# Autodesk Inventor assembly: cube sat
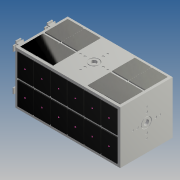
[picture p0: Inventor's stored thumbnail of the model, 180x180]
Saved by Autodesk Inventor 2017 SP1 (Build 210196100, 196)
## iProperties
Part Number: cube sat
Material: Generico
Document SubType Name: Assembly
Designer: De Grandis Leonardo
Author: De Grandis Leonardo
## Documents named in this file (8)
- E:\MATERIALE DA CARICARE\cube sat.iam
- C:\Users\Leonardo\3D Objects\struttura satellitino.ipt
- C:\Users\Leonardo\3D Objects\lente fotocamera.ipt
- C:\Users\Leonardo\3D Objects\laser 1.ipt
- C:\Users\Leonardo\3D Objects\laser 2.ipt
- C:\Users\Leonardo\3D Objects\pannello solare.ipt
- C:\Users\Leonardo\3D Objects\pannello solare_CPY.ipt
- C:\Users\Leonardo\3D Objects\pannello solare_CPY1.ipt
## Components (49 placed, 7 different names)
1. struttura satellitino:1 — Coincidente:1, Coincidente:2, Coincidente:3, Coincidente:4, Coincidente:5, Coincidente:6, Coincidente:7, Coincidente:8, Coincidente:9, Coincidente:10, Coincidente:11, Coincidente:12, Coincidente:13, Coincidente:17, Coincidente:18, Coincidente:19, Coincidente:20, Coincidente:21, Coincidente:22, Coincidente:23, Coincidente:24, Coincidente:25, Coincidente:26, Coincidente:27, Coincidente:28, Coincidente:29, Coincidente:30, Coincidente:31, Coincidente:32, Coincidente:33, Coincidente:34, Coincidente:35, Coincidente:36, Coincidente:37, Coincidente:38, Coincidente:39, Coincidente:40, Coincidente:41
2. lente fotocamera:1 — Coincidente:3
3. laser 1:1 — Coincidente:4, Coincidente:5
4. laser 1:2 — Coincidente:6, Coincidente:7
5. laser 2:1 — Coincidente:8, Coincidente:9
6. pannello solare:1 — Coincidente:10, Coincidente:11, Coincidente:12, Coincidente:13
7. pannello solare:2 — Coincidente:17, Coincidente:18, Coincidente:19
8. pannello solare:3
9. pannello solare:4
10. pannello solare:5
11. pannello solare:6
12. pannello solare:7
13. pannello solare:8
14. pannello solare:9
15. pannello solare:10
16. pannello solare:11
17. pannello solare:12
18. pannello solare_CPY:1 — Coincidente:20, Coincidente:22, Coincidente:23
19. pannello solare_CPY:2 — Coincidente:24, Coincidente:25
20. pannello solare_CPY:3
21. pannello solare_CPY:4 — Coincidente:21
22. pannello solare_CPY:5
23. pannello solare_CPY:6
24. pannello solare_CPY:7
25. pannello solare_CPY:8
26. pannello solare_CPY:9
27. pannello solare_CPY:10
28. pannello solare_CPY:11
29. pannello solare_CPY:12
30. pannello solare_CPY1:1
31. pannello solare_CPY1:2
32. pannello solare_CPY1:3
33. pannello solare_CPY1:4
34. pannello solare_CPY1:5
35. pannello solare_CPY1:6
36. pannello solare_CPY1:7
37. pannello solare_CPY1:8
38. pannello solare_CPY1:9
39. pannello solare_CPY1:10 — Coincidente:31
40. pannello solare_CPY1:11 — Coincidente:27, Coincidente:29, Coincidente:30
41. pannello solare_CPY1:12 — Coincidente:26, Coincidente:28
42. pannello solare:16 — Coincidente:32, Coincidente:33
43. pannello solare:15 — Coincidente:34, Coincidente:35
44. pannello solare:13 — Coincidente:36, Coincidente:37, Coincidente:38
45. pannello solare:17 — Coincidente:39, Coincidente:40, Coincidente:41
46. pannello solare:18
47. pannello solare:19
48. pannello solare:20
49. pannello solare:21
## Component patterns: (6 elements, first: pannello solare:1 + pannello solare:2), (6 elements, first: pannello solare_CPY:1 + pannello solare_CPY:2), (6 elements, first: pannello solare_CPY1:1 + pannello solare_CPY1:2), (2 elements, first: pannello solare:16 + pannello solare:15 + pannello solare:13 + pannello solare:17)
## Relationships (38: Mate 38)
- Coincidente:1 [Mate]: struttura satellitino:1
- Coincidente:2 [Mate]: struttura satellitino:1
- Coincidente:3 [Mate]: struttura satellitino:1 ↔ lente fotocamera:1
- Coincidente:4 [Mate]: struttura satellitino:1 ↔ laser 1:1
- Coincidente:5 [Mate]: struttura satellitino:1 ↔ laser 1:1
- Coincidente:6 [Mate]: struttura satellitino:1 ↔ laser 1:2
- Coincidente:7 [Mate]: struttura satellitino:1 ↔ laser 1:2
- Coincidente:8 [Mate]: struttura satellitino:1 ↔ laser 2:1
- Coincidente:9 [Mate]: struttura satellitino:1 ↔ laser 2:1
- Coincidente:10 [Mate]: struttura satellitino:1 ↔ pannello solare:1
- Coincidente:11 [Mate]: struttura satellitino:1 ↔ pannello solare:1
- Coincidente:12 [Mate]: struttura satellitino:1 ↔ pannello solare:1
- Coincidente:13 [Mate]: struttura satellitino:1 ↔ pannello solare:1
- Coincidente:17 [Mate]: struttura satellitino:1 ↔ pannello solare:2
- Coincidente:18 [Mate]: struttura satellitino:1 ↔ pannello solare:2
- Coincidente:19 [Mate]: struttura satellitino:1 ↔ pannello solare:2
- Coincidente:20 [Mate]: struttura satellitino:1 ↔ pannello solare_CPY:1
- Coincidente:21 [Mate]: struttura satellitino:1 ↔ pannello solare_CPY:4
- Coincidente:22 [Mate]: struttura satellitino:1 ↔ pannello solare_CPY:1
- Coincidente:23 [Mate]: struttura satellitino:1 ↔ pannello solare_CPY:1
- Coincidente:24 [Mate]: struttura satellitino:1 ↔ pannello solare_CPY:2
- Coincidente:25 [Mate]: struttura satellitino:1 ↔ pannello solare_CPY:2
- Coincidente:26 [Mate]: struttura satellitino:1 ↔ pannello solare_CPY1:12
- Coincidente:27 [Mate]: struttura satellitino:1 ↔ pannello solare_CPY1:11
- Coincidente:28 [Mate]: struttura satellitino:1 ↔ pannello solare_CPY1:12
- Coincidente:29 [Mate]: struttura satellitino:1 ↔ pannello solare_CPY1:11
- Coincidente:30 [Mate]: struttura satellitino:1 ↔ pannello solare_CPY1:11
- Coincidente:31 [Mate]: struttura satellitino:1 ↔ pannello solare_CPY1:10
- Coincidente:32 [Mate]: struttura satellitino:1 ↔ pannello solare:16
- Coincidente:33 [Mate]: struttura satellitino:1 ↔ pannello solare:16
- Coincidente:34 [Mate]: struttura satellitino:1 ↔ pannello solare:15
- Coincidente:35 [Mate]: struttura satellitino:1 ↔ pannello solare:15
- Coincidente:36 [Mate]: struttura satellitino:1 ↔ pannello solare:13
- Coincidente:37 [Mate]: struttura satellitino:1 ↔ pannello solare:13
- Coincidente:38 [Mate]: struttura satellitino:1 ↔ pannello solare:13
- Coincidente:39 [Mate]: struttura satellitino:1 ↔ pannello solare:17
- Coincidente:40 [Mate]: struttura satellitino:1 ↔ pannello solare:17
- Coincidente:41 [Mate]: struttura satellitino:1 ↔ pannello solare:17
